# Autodesk Inventor assembly: Pancake_Catch Assy
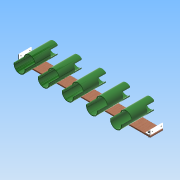
[picture p0: Inventor's stored thumbnail of the model, 180x180]
Saved by Autodesk Inventor 2018.1 (Build 221171000, 171)
## iProperties
Created: 2019-02-21
Part Number: Pancake_Catch Assy
Document SubType Name: Assembly
Designer: James
Author: James
## Documents named in this file (7)
- C:\Users\admin\Desktop\Ball Sorting Machine\Ball-Sorting-Machine\Pancake Sort\Pancake_Drop Assy.iam
- C:\Users\admin\Desktop\Ball Sorting Machine\Ball-Sorting-Machine\Pancake Sort\Nyloc Nut - M4.ipt
- C:\Users\admin\Desktop\Ball Sorting Machine\Ball-Sorting-Machine\Pancake Sort\Socket Csk Screw - (A2) - M4 x  16.ipt
- C:\Users\admin\Desktop\Ball Sorting Machine\Ball-Sorting-Machine\Pancake Sort\Pancake_Angle Bracket.ipt
- C:\Users\admin\Desktop\Ball Sorting Machine\Ball-Sorting-Machine\Pancake Sort\Socket Cap Screw - Standard - (A2) - M4 x 16.ipt
- C:\Users\admin\Desktop\Ball Sorting Machine\Ball-Sorting-Machine\Pancake Sort\Pancake_Drop Backboard.ipt
- C:\Users\admin\Desktop\Ball Sorting Machine\Ball-Sorting-Machine\Pancake Sort\Pancake_Drop Pipe.ipt
## Components (36 placed, 6 different names)
1. Pancake_Drop Backboard:1 — Flush:1, Flush:2, Flush:3, Tangent:1, Mate:33, Mate:34, Mate:35, Mate:36, Flush:9, Mate:37, Mate:38, Mate:45, Mate:46, Mate:47, Mate:48, Mate:49, Flush:10, Mate:56, Mate:59, Mate:60, Mate:61, Mate:62, Flush:11
2. Pancake_Angle Bracket:2 — Mate:45, Mate:46, Mate:47, Flush:10
3. Nyloc Nut - M4:17 — Mate:48
4. Socket Cap Screw - Standard - (A2) - M4 x 16:3
5. Nyloc Nut - M4:18 — Mate:49
6. Socket Cap Screw - Standard - (A2) - M4 x 16:4
7. Pancake_Angle Bracket:3 — Mate:56, Mate:61, Mate:62, Flush:11
8. Nyloc Nut - M4:19 — Mate:59
9. Socket Cap Screw - Standard - (A2) - M4 x 16:5
10. Nyloc Nut - M4:20 — Mate:60
11. Socket Cap Screw - Standard - (A2) - M4 x 16:6
12. Socket Csk Screw - (A2) - M4 x  16:3 — Mate:35, Flush:9
13. Nyloc Nut - M4:15 — Mate:37
14. Pancake_Drop Pipe:2 — Tangent:1, Mate:33, Mate:34, Angle:1
15. Socket Csk Screw - (A2) - M4 x  16:4 — Mate:36
16. Nyloc Nut - M4:16 — Mate:38
17. Socket Csk Screw - (A2) - M4 x  16:5
18. Nyloc Nut - M4:21
19. Pancake_Drop Pipe:3
20. Socket Csk Screw - (A2) - M4 x  16:6
21. Nyloc Nut - M4:22
22. Socket Csk Screw - (A2) - M4 x  16:7
23. Nyloc Nut - M4:23
24. Pancake_Drop Pipe:4
25. Socket Csk Screw - (A2) - M4 x  16:8
26. Nyloc Nut - M4:24
27. Socket Csk Screw - (A2) - M4 x  16:9
28. Nyloc Nut - M4:25
29. Pancake_Drop Pipe:5
30. Socket Csk Screw - (A2) - M4 x  16:10
31. Nyloc Nut - M4:26
32. Socket Csk Screw - (A2) - M4 x  16:11
33. Nyloc Nut - M4:27
34. Pancake_Drop Pipe:6
35. Socket Csk Screw - (A2) - M4 x  16:12
36. Nyloc Nut - M4:28
## Component patterns: (5 elements, first: Socket Csk Screw - (A2) - M4 x  16:3 + Nyloc Nut - M4:15 + Pancake_Drop Pipe:2 + Socket Csk Screw - (A2) - M4 x  16:4 + Nyloc Nut - M4:16)
## Relationships (39: Mate 30, Flush 7, Tangent 1, Angle 1)
- Flush:1: Pancake_Drop Backboard:1
- Flush:2: Pancake_Drop Backboard:1
- Flush:3: Pancake_Drop Backboard:1
- [Flush]: Socket Csk Screw - (A2) - M4 x  16:3 ↔ Socket Csk Screw - (A2) - M4 x  16:4
- [Mate]: Socket Csk Screw - (A2) - M4 x  16:4 ↔ Nyloc Nut - M4:16
- [Mate]: Socket Csk Screw - (A2) - M4 x  16:3 ↔ Nyloc Nut - M4:15
- Tangent:1: Pancake_Drop Backboard:1 ↔ Pancake_Drop Pipe:2
- Mate:33: Pancake_Drop Backboard:1 ↔ Pancake_Drop Pipe:2
- Mate:34: Pancake_Drop Backboard:1 ↔ Pancake_Drop Pipe:2
- Angle:1 (0 deg): Pancake_Drop Pipe:2
- Mate:35: Pancake_Drop Backboard:1 ↔ Socket Csk Screw - (A2) - M4 x  16:3
- Mate:36: Pancake_Drop Backboard:1 ↔ Socket Csk Screw - (A2) - M4 x  16:4
- Flush:9 (-5 mm): Pancake_Drop Backboard:1 ↔ Socket Csk Screw - (A2) - M4 x  16:3
- Mate:37: Pancake_Drop Backboard:1 ↔ Nyloc Nut - M4:15
- Mate:38: Pancake_Drop Backboard:1 ↔ Nyloc Nut - M4:16
- [Mate]: Pancake_Angle Bracket:2 ↔ Socket Cap Screw - Standard - (A2) - M4 x 16:3
- [Mate]: Pancake_Angle Bracket:2 ↔ Socket Cap Screw - Standard - (A2) - M4 x 16:4
- [Mate]: Pancake_Angle Bracket:2 ↔ Socket Cap Screw - Standard - (A2) - M4 x 16:3
- [Mate]: Pancake_Angle Bracket:2 ↔ Socket Cap Screw - Standard - (A2) - M4 x 16:4
- [Mate]: Socket Cap Screw - Standard - (A2) - M4 x 16:3 ↔ Nyloc Nut - M4:18
- [Mate]: Nyloc Nut - M4:17 ↔ Socket Cap Screw - Standard - (A2) - M4 x 16:4
- Mate:45: Pancake_Drop Backboard:1 ↔ Pancake_Angle Bracket:2
- Mate:46: Pancake_Drop Backboard:1 ↔ Pancake_Angle Bracket:2
- Mate:47: Pancake_Drop Backboard:1 ↔ Pancake_Angle Bracket:2
- Mate:48: Pancake_Drop Backboard:1 ↔ Nyloc Nut - M4:17
- Mate:49: Pancake_Drop Backboard:1 ↔ Nyloc Nut - M4:18
- Flush:10: Pancake_Drop Backboard:1 ↔ Pancake_Angle Bracket:2
- [Mate]: Pancake_Angle Bracket:3 ↔ Socket Cap Screw - Standard - (A2) - M4 x 16:5
- [Mate]: Pancake_Angle Bracket:3 ↔ Socket Cap Screw - Standard - (A2) - M4 x 16:6
- [Mate]: Pancake_Angle Bracket:3 ↔ Socket Cap Screw - Standard - (A2) - M4 x 16:5
- [Mate]: Pancake_Angle Bracket:3 ↔ Socket Cap Screw - Standard - (A2) - M4 x 16:6
- [Mate]: Socket Cap Screw - Standard - (A2) - M4 x 16:5 ↔ Nyloc Nut - M4:20
- [Mate]: Nyloc Nut - M4:19 ↔ Socket Cap Screw - Standard - (A2) - M4 x 16:6
- Mate:56: Pancake_Drop Backboard:1 ↔ Pancake_Angle Bracket:3
- Mate:59: Pancake_Drop Backboard:1 ↔ Nyloc Nut - M4:19
- Mate:60: Pancake_Drop Backboard:1 ↔ Nyloc Nut - M4:20
- Mate:61: Pancake_Drop Backboard:1 ↔ Pancake_Angle Bracket:3
- Mate:62: Pancake_Drop Backboard:1 ↔ Pancake_Angle Bracket:3
- Flush:11: Pancake_Drop Backboard:1 ↔ Pancake_Angle Bracket:3
## Named parameters: d47_d9 = 0 mm, d48_d12 = 0 mm, d49_d13 = 0 mm, d59_d39 = 0 mm, d60_d40 = 0 mm, d61_d41 = 0 mm, d62_d42 = 0 mm, d63_d45 = 0 mm, d64_d46 = 0 mm, d71_d59_d39 = 0 mm, d72_d60_d40 = 0 mm, d73_d61_d41 = 0 mm, d74_d62_d42 = 0 mm, d75_d63_d45 = 0 mm, d76_d64_d46 = 0 mm
